# Autodesk Inventor assembly: with movable rod
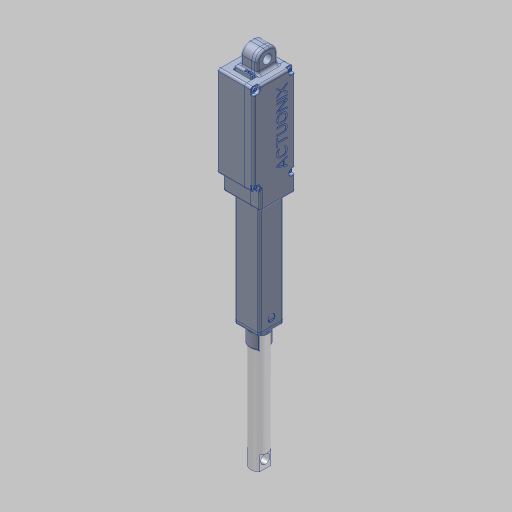
[picture p0: Inventor's stored thumbnail of the model, 512x512]
Saved by Autodesk Inventor 2023.5 (Build 275446000, 446)
## iProperties
Created: 2025-01-30
Part Number: with movable rod
Document SubType Name: Assembly
Designer: slick
Author: slick
## Documents named in this file (3)
- C:\Users\slick\OneDrive\Desktop\2025-ReefScape---CAD\COMMON PARTS\Z - STEPS\WCP-0407-Retracted\with movable rod.iam
- C:\Users\slick\OneDrive\Desktop\2025-ReefScape---CAD\COMMON PARTS\Z - STEPS\WCP-0407-Retracted\WCP-0407-Retracted.ipt
- C:\Users\slick\OneDrive\Desktop\2025-ReefScape---CAD\COMMON PARTS\Z - STEPS\WCP-0407-Retracted\rod.ipt
## Components (2 placed, 2 different names)
1. WCP-0407-Retracted:1 — Flush:2
2. rod:1 — Flush:1, Mate:1, Flush:2
## Relationships (3: Flush 2, Mate 1)
- Flush:1: rod:1
- Mate:1: rod:1
- Flush:2: WCP-0407-Retracted:1 ↔ rod:1
